# Autodesk Inventor assembly: tower_MIR
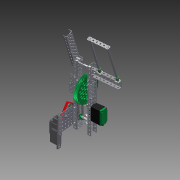
[picture p0: Inventor's stored thumbnail of the model, 180x180]
Saved by Autodesk Inventor 2014 SP1 (Build 180222100, 222)
## iProperties
Created: 2014-03-19
Part Number: tower_MIR
Document SubType Name: Assembly
Designer: Ryan
Author: Ryan
## Documents named in this file (30)
- C:\Users\Ryan\Desktop\sw\toss up 5th A bot\tower\tower_MIR.iam
- C:\Users\Ryan\Desktop\sw\lib\Aperture VEX CAD Library\Metal\C Channel\2 x 18.ipt
- C:\Users\Ryan\Desktop\sw\lib\Aperture VEX CAD Library\Bearing Blocks\Bearing Block.ipt
- C:\Users\Ryan\Desktop\sw\lib\Aperture VEX CAD Library\Hardware\8-32\8-32_.500.ipt
- C:\Users\Ryan\Desktop\sw\lib\Aperture VEX CAD Library\Hardware\8-32\8-32 nylock.ipt
- C:\Users\Ryan\Desktop\sw\lib\Aperture VEX CAD Library\Motors\2-Wire Motor 393-Without Wire.iam
- C:\Users\Ryan\Desktop\sw\lib\Aperture VEX CAD Library\Hardware\6-32\6-32_.250.ipt
- C:\Users\Ryan\Desktop\sw\lib\Aperture VEX CAD Library\Spacers\thin\SPACER-0320-0125.ipt
- C:\Users\Ryan\Desktop\sw\lib\Aperture VEX CAD Library\Gears\High Strength Gears\HS-GEAR-12TOOTH.ipt
- C:\Users\Ryan\Desktop\sw\lib\Aperture VEX CAD Library\Gears\High Strength Gears\Green HS 84.iam
- C:\Users\Ryan\Desktop\sw\lib\Aperture VEX CAD Library\Spacers\thin\SPACER-0320-0250.ipt
- C:\Users\Ryan\Desktop\sw\lib\Aperture VEX CAD Library\Hardware\Shaft Collar.ipt
- C:\Users\Ryan\Desktop\sw\lib\Aperture VEX CAD Library\Spacers\thin\SPACER-0320-00625.ipt
- C:\Users\Ryan\Desktop\sw\lib\Aperture VEX CAD Library\Standoffs\BEAM-0500.ipt
- C:\Users\Ryan\Desktop\sw\toss up 5th A bot\tower\large ball knocker right_MIR.iam
- C:\Users\Ryan\Desktop\sw\lib\Aperture VEX CAD Library\Metal\L Bar\2 x 4.ipt
- C:\Users\Ryan\Desktop\sw\lib\Aperture VEX CAD Library\Hardware\8-32\8-32_1.500.ipt
- C:\Users\Ryan\Desktop\sw\lib\Aperture VEX CAD Library\Hardware\8-32\8-32_.375.ipt
- C:\Users\Ryan\Desktop\sw\lib\Aperture VEX CAD Library\Metal\Plate\2 x 5.ipt
- C:\Users\Ryan\Desktop\sw\lib\Aperture VEX CAD Library\Hardware\8-32\8-23_.750.ipt
- C:\Users\Ryan\Desktop\sw\lib\Aperture VEX CAD Library\Spacers\SPACER-0500-0125.ipt
- C:\Users\Ryan\Desktop\sw\lib\Aperture VEX CAD Library\Spacers\thin\SPACER-0320-0375.ipt
- C:\Users\Ryan\Desktop\sw\lib\Aperture VEX CAD Library\Metal\C Channel\2 x 10.ipt
- C:\Users\Ryan\Desktop\sw\lib\Aperture VEX CAD Library\Metal\C Channel\5 x 5.ipt
- C:\Users\Ryan\Desktop\sw\lib\Super Sonic Sparks VEX CAD Library\Motors & Sensors\Optical Shaft (Quadrature) Encoder.iam
- C:\Users\Ryan\Desktop\sw\lib\Super Sonic Sparks VEX CAD Library\Gears & Pulleys\12-Tooth Sprocket - Cut.ipt
- C:\Users\Ryan\Desktop\sw\lib\Super Sonic Sparks VEX CAD Library\Gears & Pulleys\12-Tooth Sprocket.ipt
- C:\Users\Ryan\Desktop\sw\toss up 5th A bot\tower\tower_MIR\Design Accelerator\V-Belt transmission1.iam
- C:\Users\Ryan\Desktop\sw\lib\Super Sonic Sparks VEX CAD Library\Chain & Tank Tread\Chain Link.ipt
- C:\Users\Ryan\Desktop\sw\lib\Super Sonic Sparks VEX CAD Library\Other Parts\Power Expander.iam
## Components (132 placed, 29 different names)
1. 2 x 18:1 — Mate:1, Mate:5, Mate:4, Mate:3, Mate:9, Mate:8, Mate:7, Mate:6, Mate:13, Mate:12, Mate:11, Mate:10, Mate:15, Mate:17, Mate:26, Mate:36, Mate:35, Mate:34, Mate:33, Mate:46, Mate:37, Mate:39, Mate:48, Flush:8, Flush:7, Flush:6, Flush:9, Mate:87, Flush:12, Flush:11, Mate:91, Flush:14, Flush:13, Mate:92, Mate:134, Mate:150, Mate:151, Mate:152, Mate:153, Mate:156
2. Bearing Block:1 — Mate:1, Mate:5, Mate:4, Mate:3, Mate:14, Mate:16, Mate:18, Mate:21, Mate:71, Mate:88, Mate:94, Mate:93
3. Bearing Block:2 — Mate:9, Mate:8, Mate:7, Mate:6, Mate:22, Mate:23, Mate:31, Mate:32, Mate:40
4. Bearing Block:3 — Mate:13, Mate:12, Mate:11, Mate:10, Mate:24, Mate:25, Mate:38
5. 8-32_.500:1 — Mate:15, Mate:14, Mate:19
6. 8-32_.500:2 — Mate:17, Mate:16, Mate:20, Mate:74
7. 8-32 nylock:1 — Mate:19, Mate:18
8. 8-32 nylock:2 — Mate:21, Mate:20
9. 8-32_.500:3 — Mate:26, Mate:22, Flush:3, Mate:27
10. 8-32_.500:4 — Flush:3, Mate:23, Flush:2, Mate:28
11. 8-32_.500:5 — Flush:2, Mate:24, Flush:1, Mate:29
12. 8-32_.500:6 — Flush:1, Mate:25, Mate:30
13. 8-32 nylock:3 — Mate:31, Mate:27
14. 8-32 nylock:4 — Mate:28, Flush:4, Mate:80
15. 8-32 nylock:5 — Mate:32, Flush:4, Mate:29, Flush:5
16. 8-32 nylock:6 — Flush:5, Mate:30
17. 2-Wire Motor 393-Without Wire:1 [sub-assembly] — Mate:36, Mate:35, Mate:34, Mate:33, Mate:45, Mate:47
18. 6-32_.250:1 — Mate:46, Mate:45
19. SPACER-0320-0125:1 — Mate:38, Mate:37, Mate:42, Mate:41, Mate:144
20. SPACER-0320-0125:2 — Mate:40, Mate:39, Mate:44, Mate:43
21. HS-GEAR-12TOOTH:1 — Mate:42, Mate:41
22. Green HS 84:1 [sub-assembly] — Mate:44, Mate:43, Mate:51, Mate:76
23. 6-32_.250:2 — Mate:48, Mate:47
24. 2 x 18:2 — Flush:8, Flush:7, Flush:6, Mate:55, Mate:72, Mate:77, Mate:75, Mate:73, Mate:78, Mate:83, Flush:16, Flush:15, Mate:102, Mate:103, Mate:106, Mate:110, Mate:112, Mate:123, Mate:124, Mate:122, Mate:131, Mate:136, Mate:138, Flush:17, Flush:18, Mate:142, Mate:143, Mate:145, Mate:162
25. SPACER-0320-0250:1 — Mate:51, Mate:54, Mate:53, Mate:57, Mate:56
26. Shaft Collar:1 — Mate:55, Mate:54, Mate:53
27. SPACER-0320-00625:1 — Mate:57, Mate:56
28. Shaft Collar:2 — Mate:144, Mate:146, Mate:147, Mate:148, Mate:149
29. Bearing Block:4 — Mate:72, Mate:71, Mate:60, Mate:61, Mate:63, Mate:64, Mate:82, Mate:81, Mate:84
30. Bearing Block:5 — Mate:77, Mate:76, Mate:66, Mate:67, Mate:68, Mate:79
31. 8-32_.500:7 — Mate:75, Mate:60, Mate:62
32. 8-32_.500:8 — Mate:74, Mate:73, Mate:61, Mate:65
33. 8-32 nylock:7 — Mate:63, Mate:62
34. 8-32 nylock:8 — Mate:65, Mate:64
35. 8-32_.500:9 — Mate:66, Flush:10, Mate:69
36. 8-32_.500:10 — Mate:78, Mate:67, Flush:10, Mate:70
37. 8-32 nylock:9 — Mate:69, Mate:68
38. 8-32 nylock:10 — Mate:80, Mate:79, Mate:70
39. SPACER-0320-0125:3 — Mate:82, Mate:81, Mate:96
40. 8-32 nylock:11 — Mate:84, Mate:83, Mate:86, Mate:85
41. SPACER-0320-0125:4 — Mate:86, Mate:85, Mate:95
42. BEAM-0500:1 — Mate:88, Mate:87, Mate:90, Mate:89
43. SPACER-0320-0125:5 — Mate:90, Mate:89
44. large ball knocker right_MIR:1 [sub-assembly] — Flush:12, Flush:11, Mate:91, Angle:1
45. 2 x 4:1 — Flush:14, Flush:13, Mate:92, Mate:99, Mate:98, Mate:97, Mate:101, Mate:135, Mate:133, Mate:137
46. 8-32_.500:11 — Mate:94, Mate:93
47. 8-32_1.500:1 — Mate:96, Mate:95
48. 8-32 nylock:12 — Mate:99, Mate:98, Mate:97, Mate:100
49. 8-32_.375:1 — Mate:101, Mate:100
50. 2 x 5:1 — Flush:16, Flush:15, Mate:102, Mate:105, Mate:104, Mate:108, Mate:107, Mate:114, Mate:113, Mate:136
51. 8-32_.375:2 — Mate:105, Mate:104, Mate:103, Mate:111
52. 8-32_.375:3 — Mate:108, Mate:107, Mate:106, Mate:109
53. 8-32 nylock:13 — Mate:110, Mate:109
54. 8-32 nylock:14 — Mate:112, Mate:111
55. 8-23_.750:1 — Mate:114, Mate:113, Mate:115, Mate:117, Mate:116, Mate:118
56. BEAM-0500:2 — Mate:115, Mate:137, Mate:119
57. SPACER-0500-0125:1 — Mate:137, Mate:117, Mate:116
58. 8-32 nylock:15 — Mate:136, Mate:119, Mate:118
59. SPACER-0320-0375:1 — Mate:123, Mate:121, Mate:120, Mate:127, Mate:126, Mate:125, Mate:128
60. SPACER-0320-0250:2 — Mate:124, Mate:122, Mate:121, Mate:120, Mate:130
61. 2 x 10:1 — Mate:127, Mate:126, Mate:125, Mate:129, Angle:1
62. 8-32_.375:4 — Mate:129, Mate:128
63. 8-32 nylock:16 — Mate:131, Mate:130
64. 5 x 5:1 — Mate:138, Flush:17, Flush:18, Mate:140, Mate:141, Mate:165, Mate:167, Mate:168, Mate:170, Mate:173, Mate:174, Flush:176
65. Optical Shaft (Quadrature) Encoder:1 [sub-assembly] — Mate:164, Mate:165, Mate:169
66. 12-Tooth Sprocket - Cut:1 — Mate:145, Mate:146, Mate:147, Mate:171, Mate:172, Flush:19
67. SPACER-0320-00625:2 — Mate:148, Mate:149
68. SPACER-0320-0375:2 — Mate:158, Mate:159, Mate:160, Mate:161
69. Shaft Collar:3 — Mate:160, Mate:161, Mate:163
70. 12-Tooth Sprocket:1 — Mate:162, Mate:163, Mate:164
71. 8-32_.500:14 — Mate:167, Mate:168, Mate:169
72. 8-32 nylock:23 — Mate:170
73. V-Belt transmission:1 [sub-assembly]
74. Power Expander:1 [sub-assembly] — Mate:173, Mate:174, Flush:176
75. 8-32 nylock:17 — Mate:135, Mate:132
76. 8-32_.375:5 — Mate:134, Mate:133, Mate:132, Mate:137
77. 8-32 nylock:18
78. 8-32_.375:6
79. 8-32_.375:7 — Mate:140, Mate:141, Mate:143
80. 8-32 nylock:19 — Mate:142
81. 8-32_.375:8
82. 8-32 nylock:20
83. Bearing Block:6 — Mate:150, Mate:151, Mate:152, Mate:153, Mate:155, Mate:157, Mate:158, Mate:159
84. Bearing Block:7
85. Chain Link:1 — Mate:171, Mate:172, Flush:19
86. Chain Link:2
87. Chain Link:3
88. Chain Link:4
89. Chain Link:5
90. Chain Link:6
91. Chain Link:7
92. Chain Link:8
93. Chain Link:9
94. Chain Link:10
95. Chain Link:11
96. Chain Link:12
97. Chain Link:13
98. Chain Link:14
99. Chain Link:15
100. Chain Link:16
101. Chain Link:17
102. Chain Link:18
103. Chain Link:19
104. Chain Link:20
105. Chain Link:21
106. Chain Link:22
107. Chain Link:23
108. Chain Link:24
109. Chain Link:25
110. Chain Link:26
111. Chain Link:27
112. Chain Link:28
113. Chain Link:29
114. Chain Link:30
115. Chain Link:31
116. Chain Link:32
117. Chain Link:33
118. Chain Link:34
119. Chain Link:35
120. Chain Link:36
121. Chain Link:37
122. Chain Link:38
123. Chain Link:39
124. Chain Link:40
125. 8-32 nylock:21 — Mate:157
126. 8-32_.500:12 — Mate:155, Mate:156
127. 8-32 nylock:22
128. 8-32_.500:13
129. 8-32 nylock:24
130. 8-32_.500:15
131. 8-32 nylock:25
132. 8-32_.500:16
## Component patterns: (2 elements, first: 8-32 nylock:17 + 8-32_.375:5), (2 elements, first: 8-32_.375:7 + 8-32 nylock:19), (2 elements, first: Bearing Block:6), (40 elements, first: Chain Link:1), (2 elements, first: 8-32 nylock:21 + 8-32_.500:12), Component Pattern 3:2 (2 elements)
## Relationships (191: Mate 170, Flush 20, Angle 1)
- Mate:1: 2 x 18:1 ↔ Bearing Block:1
- Mate:5 (2.3114 mm): 2 x 18:1 ↔ Bearing Block:1
- Mate:4 (2.3114 mm): 2 x 18:1 ↔ Bearing Block:1
- Mate:3 (2.3114 mm): 2 x 18:1 ↔ Bearing Block:1
- Mate:9 (2.3114 mm): 2 x 18:1 ↔ Bearing Block:2
- Mate:8 (2.3114 mm): 2 x 18:1 ↔ Bearing Block:2
- Mate:7 (2.3114 mm): 2 x 18:1 ↔ Bearing Block:2
- Mate:6: 2 x 18:1 ↔ Bearing Block:2
- Mate:13 (2.3114 mm): 2 x 18:1 ↔ Bearing Block:3
- Mate:12 (2.3114 mm): 2 x 18:1 ↔ Bearing Block:3
- Mate:11: 2 x 18:1 ↔ Bearing Block:3
- Mate:10 (2.3114 mm): 2 x 18:1 ↔ Bearing Block:3
- Mate:15: 2 x 18:1 ↔ 8-32_.500:1
- Mate:14: Bearing Block:1 ↔ 8-32_.500:1
- Mate:17: 2 x 18:1 ↔ 8-32_.500:2
- Mate:16: Bearing Block:1 ↔ 8-32_.500:2
- Mate:19: 8-32_.500:1 ↔ 8-32 nylock:1
- Mate:18: Bearing Block:1 ↔ 8-32 nylock:1
- Mate:21: Bearing Block:1 ↔ 8-32 nylock:2
- Mate:20: 8-32_.500:2 ↔ 8-32 nylock:2
- Mate:26: 2 x 18:1 ↔ 8-32_.500:3
- Mate:22: Bearing Block:2 ↔ 8-32_.500:3
- Flush:3: 8-32_.500:3 ↔ 8-32_.500:4
- Mate:23: Bearing Block:2 ↔ 8-32_.500:4
- Flush:2: 8-32_.500:4 ↔ 8-32_.500:5
- Mate:24: Bearing Block:3 ↔ 8-32_.500:5
- Flush:1: 8-32_.500:5 ↔ 8-32_.500:6
- Mate:25: Bearing Block:3 ↔ 8-32_.500:6
- Mate:31: Bearing Block:2 ↔ 8-32 nylock:3
- Mate:27: 8-32_.500:3 ↔ 8-32 nylock:3
- Mate:28: 8-32_.500:4 ↔ 8-32 nylock:4
- Mate:32: Bearing Block:2 ↔ 8-32 nylock:5
- Flush:4: 8-32 nylock:4 ↔ 8-32 nylock:5
- Mate:29: 8-32_.500:5 ↔ 8-32 nylock:5
- Flush:5: 8-32 nylock:5 ↔ 8-32 nylock:6
- Mate:30: 8-32_.500:6 ↔ 8-32 nylock:6
- Mate:36 (2.3114 mm): 2 x 18:1 ↔ 2-Wire Motor 393-Without Wire:1
- Mate:35 (2.3114 mm): 2 x 18:1 ↔ 2-Wire Motor 393-Without Wire:1
- Mate:34 (2.3114 mm): 2 x 18:1 ↔ 2-Wire Motor 393-Without Wire:1
- Mate:33: 2 x 18:1 ↔ 2-Wire Motor 393-Without Wire:1
- Mate:46: 2 x 18:1 ↔ 6-32_.250:1
- Mate:45: 2-Wire Motor 393-Without Wire:1 ↔ 6-32_.250:1
- Mate:38: Bearing Block:3 ↔ SPACER-0320-0125:1
- Mate:37: 2 x 18:1 ↔ SPACER-0320-0125:1
- Mate:40: Bearing Block:2 ↔ SPACER-0320-0125:2
- Mate:39: 2 x 18:1 ↔ SPACER-0320-0125:2
- Mate:42: SPACER-0320-0125:1 ↔ HS-GEAR-12TOOTH:1
- Mate:41: SPACER-0320-0125:1 ↔ HS-GEAR-12TOOTH:1
- Mate:44: SPACER-0320-0125:2 ↔ Green HS 84:1
- Mate:43: SPACER-0320-0125:2 ↔ Green HS 84:1
- Mate:48: 2 x 18:1 ↔ 6-32_.250:2
- Mate:47: 2-Wire Motor 393-Without Wire:1 ↔ 6-32_.250:2
- Flush:8 (50.8 mm): 2 x 18:1 ↔ 2 x 18:2
- Flush:7: 2 x 18:1 ↔ 2 x 18:2
- Flush:6: 2 x 18:1 ↔ 2 x 18:2
- Mate:51: Green HS 84:1 ↔ SPACER-0320-0250:1
- Mate:55: 2 x 18:2 ↔ Shaft Collar:1
- Mate:54: SPACER-0320-0250:1 ↔ Shaft Collar:1
- Mate:53: SPACER-0320-0250:1 ↔ Shaft Collar:1
- Mate:57: SPACER-0320-0250:1 ↔ SPACER-0320-00625:1
- Mate:56: SPACER-0320-0250:1 ↔ SPACER-0320-00625:1
- Flush:9 (17.8816 mm): 2 x 18:1
- Mate:72: 2 x 18:2 ↔ Bearing Block:4
- Mate:71: Bearing Block:1 ↔ Bearing Block:4
- Mate:77: 2 x 18:2 ↔ Bearing Block:5
- Mate:76: Green HS 84:1 ↔ Bearing Block:5
- Mate:75: 2 x 18:2 ↔ 8-32_.500:7
- Mate:60: Bearing Block:4 ↔ 8-32_.500:7
- Mate:74: 8-32_.500:2 ↔ 8-32_.500:8
- Mate:73: 2 x 18:2 ↔ 8-32_.500:8
- Mate:61: Bearing Block:4 ↔ 8-32_.500:8
- Mate:63: Bearing Block:4 ↔ 8-32 nylock:7
- Mate:62: 8-32_.500:7 ↔ 8-32 nylock:7
- Mate:65: 8-32_.500:8 ↔ 8-32 nylock:8
- Mate:64: Bearing Block:4 ↔ 8-32 nylock:8
- Mate:66: Bearing Block:5 ↔ 8-32_.500:9
- Mate:78: 2 x 18:2 ↔ 8-32_.500:10
- Mate:67: Bearing Block:5 ↔ 8-32_.500:10
- Flush:10: 8-32_.500:9 ↔ 8-32_.500:10
- Mate:69: 8-32_.500:9 ↔ 8-32 nylock:9
- Mate:68: Bearing Block:5 ↔ 8-32 nylock:9
- Mate:80: 8-32 nylock:4 ↔ 8-32 nylock:10
- Mate:79: Bearing Block:5 ↔ 8-32 nylock:10
- Mate:70: 8-32_.500:10 ↔ 8-32 nylock:10
- Mate:82: Bearing Block:4 ↔ SPACER-0320-0125:3
- Mate:81: Bearing Block:4 ↔ SPACER-0320-0125:3
- Mate:84: Bearing Block:4 ↔ 8-32 nylock:11
- Mate:83: 2 x 18:2 ↔ 8-32 nylock:11
- Mate:86: 8-32 nylock:11 ↔ SPACER-0320-0125:4
- Mate:85: 8-32 nylock:11 ↔ SPACER-0320-0125:4
- Mate:88: Bearing Block:1 ↔ BEAM-0500:1
- Mate:87: 2 x 18:1 ↔ BEAM-0500:1
- Mate:90: BEAM-0500:1 ↔ SPACER-0320-0125:5
- Mate:89: BEAM-0500:1 ↔ SPACER-0320-0125:5
- Flush:12: 2 x 18:1 ↔ large ball knocker right_MIR:1
- Flush:11: 2 x 18:1 ↔ large ball knocker right_MIR:1
- Mate:91: 2 x 18:1 ↔ large ball knocker right_MIR:1
- Flush:14: 2 x 18:1 ↔ 2 x 4:1
- Flush:13: 2 x 18:1 ↔ 2 x 4:1
- Mate:92: 2 x 18:1 ↔ 2 x 4:1
- Mate:94: Bearing Block:1 ↔ 8-32_.500:11
- Mate:93: Bearing Block:1 ↔ 8-32_.500:11
- Mate:96: SPACER-0320-0125:3 ↔ 8-32_1.500:1
- Mate:95: SPACER-0320-0125:4 ↔ 8-32_1.500:1
- Mate:99 (2.3114 mm): 2 x 4:1 ↔ 8-32 nylock:12
- Mate:98 (2.3114 mm): 2 x 4:1 ↔ 8-32 nylock:12
- Mate:97 (1.1684 mm): 2 x 4:1 ↔ 8-32 nylock:12
- Mate:101: 2 x 4:1 ↔ 8-32_.375:1
- Mate:100: 8-32 nylock:12 ↔ 8-32_.375:1
- Flush:16: 2 x 18:2 ↔ 2 x 5:1
- Flush:15: 2 x 18:2 ↔ 2 x 5:1
- Mate:102: 2 x 18:2 ↔ 2 x 5:1
- Mate:105: 2 x 5:1 ↔ 8-32_.375:2
- Mate:104 (2.3114 mm): 2 x 5:1 ↔ 8-32_.375:2
- Mate:103 (2.3114 mm): 2 x 18:2 ↔ 8-32_.375:2
- Mate:108: 2 x 5:1 ↔ 8-32_.375:3
- Mate:107 (2.3114 mm): 2 x 5:1 ↔ 8-32_.375:3
- Mate:106 (2.3114 mm): 2 x 18:2 ↔ 8-32_.375:3
- Mate:110: 2 x 18:2 ↔ 8-32 nylock:13
- Mate:109: 8-32_.375:3 ↔ 8-32 nylock:13
- Mate:112: 2 x 18:2 ↔ 8-32 nylock:14
- Mate:111: 8-32_.375:2 ↔ 8-32 nylock:14
- Mate:114 (2.3114 mm): 2 x 5:1 ↔ 8-23_.750:1
- Mate:113 (2.3114 mm): 2 x 5:1 ↔ 8-23_.750:1
- Mate:115: 8-23_.750:1 ↔ BEAM-0500:2
- Mate:137: BEAM-0500:2 ↔ SPACER-0500-0125:1
- Mate:117: 8-23_.750:1 ↔ SPACER-0500-0125:1
- Mate:116: 8-23_.750:1 ↔ SPACER-0500-0125:1
- Mate:136: 2 x 5:1 ↔ 8-32 nylock:15
- Mate:119 (1.1684 mm): BEAM-0500:2 ↔ 8-32 nylock:15
- Mate:118: 8-23_.750:1 ↔ 8-32 nylock:15
- Mate:123 (2.3114 mm): 2 x 18:2 ↔ SPACER-0320-0375:1
- Mate:124 (2.3114 mm): 2 x 18:2 ↔ SPACER-0320-0250:2
- Mate:122: 2 x 18:2 ↔ SPACER-0320-0250:2
- Mate:121: SPACER-0320-0375:1 ↔ SPACER-0320-0250:2
- Mate:120: SPACER-0320-0375:1 ↔ SPACER-0320-0250:2
- Mate:127 (2.3114 mm): SPACER-0320-0375:1 ↔ 2 x 10:1
- Mate:126 (2.3114 mm): SPACER-0320-0375:1 ↔ 2 x 10:1
- Mate:125: SPACER-0320-0375:1 ↔ 2 x 10:1
- Mate:129: 2 x 10:1 ↔ 8-32_.375:4
- Mate:128: SPACER-0320-0375:1 ↔ 8-32_.375:4
- Mate:131: 2 x 18:2 ↔ 8-32 nylock:16
- Mate:130: SPACER-0320-0250:2 ↔ 8-32 nylock:16
- Mate:135: 2 x 4:1 ↔ 8-32 nylock:17
- Mate:134: 2 x 18:1 ↔ 8-32_.375:5
- Mate:133 (2.3114 mm): 2 x 4:1 ↔ 8-32_.375:5
- Mate:132: 8-32 nylock:17 ↔ 8-32_.375:5
- Mate:136: 2 x 18:2
- Mate:137 (2.3114 mm): 2 x 4:1 ↔ 8-32_.375:5
- Mate:138: 2 x 18:2 ↔ 5 x 5:1
- Flush:17: 2 x 18:2 ↔ 5 x 5:1
- Flush:18: 2 x 18:2 ↔ 5 x 5:1
- [Mate]: 8-32_.375:7 ↔ 8-32 nylock:19
- Mate:140 (2.3114 mm): 5 x 5:1 ↔ 8-32_.375:7
- Mate:141: 5 x 5:1 ↔ 8-32_.375:7
- Mate:142: 2 x 18:2 ↔ 8-32 nylock:19
- Mate:143 (2.3114 mm): 2 x 18:2 ↔ 8-32_.375:7
- Mate:144: SPACER-0320-0125:1 ↔ Shaft Collar:2
- Mate:145: 2 x 18:2 ↔ 12-Tooth Sprocket - Cut:1
- Mate:146: Shaft Collar:2 ↔ 12-Tooth Sprocket - Cut:1
- Mate:147: Shaft Collar:2 ↔ 12-Tooth Sprocket - Cut:1
- Mate:148: Shaft Collar:2 ↔ SPACER-0320-00625:2
- Mate:149: Shaft Collar:2 ↔ SPACER-0320-00625:2
- Mate:150: 2 x 18:1 ↔ Bearing Block:6
- Mate:151 (2.3114 mm): 2 x 18:1 ↔ Bearing Block:6
- Mate:152 (2.3114 mm): 2 x 18:1 ↔ Bearing Block:6
- Mate:153 (2.3114 mm): 2 x 18:1 ↔ Bearing Block:6
- [Mate]: 8-32 nylock:21 ↔ 8-32_.500:12
- Mate:155: Bearing Block:6 ↔ 8-32_.500:12
- Mate:156: 2 x 18:1 ↔ 8-32_.500:12
- Mate:157: Bearing Block:6 ↔ 8-32 nylock:21
- Mate:158: SPACER-0320-0375:2 ↔ Bearing Block:6
- Mate:159: SPACER-0320-0375:2 ↔ Bearing Block:6
- Mate:160: SPACER-0320-0375:2 ↔ Shaft Collar:3
- Mate:161: SPACER-0320-0375:2 ↔ Shaft Collar:3
- Mate:162: 2 x 18:2 ↔ 12-Tooth Sprocket:1
- Mate:163: Shaft Collar:3 ↔ 12-Tooth Sprocket:1
- Mate:164: Optical Shaft (Quadrature) Encoder:1 ↔ 12-Tooth Sprocket:1
- Mate:165: 5 x 5:1 ↔ Optical Shaft (Quadrature) Encoder:1
- [Mate]: 8-32_.500:14 ↔ 8-32 nylock:23
- Mate:167 (2.3114 mm): 5 x 5:1 ↔ 8-32_.500:14
- Mate:168 (2.3114 mm): 5 x 5:1 ↔ 8-32_.500:14
- Mate:169: Optical Shaft (Quadrature) Encoder:1 ↔ 8-32_.500:14
- Mate:170: 5 x 5:1 ↔ 8-32 nylock:23
- Mate:171: 12-Tooth Sprocket - Cut:1 ↔ Chain Link:1
- Mate:172: 12-Tooth Sprocket - Cut:1 ↔ Chain Link:1
- Flush:19 (-3.15 mm): 12-Tooth Sprocket - Cut:1 ↔ Chain Link:1
- Mate:173: 5 x 5:1 ↔ Power Expander:1
- Mate:174 (-2.3114 mm): 5 x 5:1 ↔ Power Expander:1
- Flush:176 (-2.3114 mm): 5 x 5:1 ↔ Power Expander:1
- Angle:1 (90 deg): large ball knocker right_MIR:1 ↔ 2 x 10:1
## Named parameters: q = 2.3114 mm, d160_d123 = 0 mm, d179_d35 = 0 mm, d195_d33 = 0 mm
